# Autodesk Inventor assembly: Concept
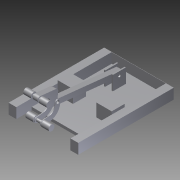
[picture p0: Inventor's stored thumbnail of the model, 180x180]
Saved by Autodesk Inventor 2012 (Build 160160000, 160)
## iProperties
Created: 2011-09-11
Part Number: Concept
Document SubType Name: Assembly
Designer: Ian Walters
Author: Ian Walters
## Documents named in this file (6)
- C:\Users\robotics\Dropbox\CAD Inventor\BunnyBot\Concept.iam
- C:\Users\robotics\Dropbox\CAD Inventor\BunnyBot\Base.ipt
- C:\Users\robotics\Dropbox\CAD Inventor\BunnyBot\Arm.ipt
- C:\Users\robotics\Dropbox\CAD Inventor\BunnyBot\Claw.ipt
- C:\Users\robotics\Dropbox\CAD Inventor\BunnyBot\Roller.ipt
- C:\Users\robotics\Dropbox\CAD Inventor\BunnyBot\Plunger.ipt
## Components (7 placed, 5 different names)
1. Base:1 — Flush:1, Flush:2, Flush:3, Mate:1, Mate:2
2. Arm:1 — Mate:1, Mate:2, Insert:1, Insert:2, Mate:5, Mate:7, Mate:8
3. Claw:1 — Insert:1, Mate:3, Mate:4, Mate:6
4. Claw:2 — Insert:2, Mate:3
5. Roller:1 — Mate:5, Mate:7
6. Roller:2 — Mate:4, Mate:6
7. Plunger:1 — Mate:8
## Relationships (13: Mate 8, Flush 3, Insert 2)
- Flush:1: Base:1
- Flush:2: Base:1
- Flush:3: Base:1
- Mate:1: Base:1 ↔ Arm:1
- Mate:2 (6.35 mm): Base:1 ↔ Arm:1
- Insert:1: Arm:1 ↔ Claw:1
- Insert:2: Arm:1 ↔ Claw:2
- Mate:3: Claw:1 ↔ Claw:2
- Mate:4: Claw:1 ↔ Roller:2
- Mate:5: Arm:1 ↔ Roller:1
- Mate:6 (6.35 mm): Claw:1 ↔ Roller:2
- Mate:7 (12.7 mm): Arm:1 ↔ Roller:1
- Mate:8: Arm:1 ↔ Plunger:1
